# Autodesk Inventor assembly: A-02-0
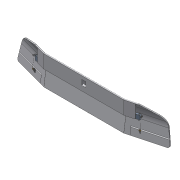
[picture p0: Inventor's stored thumbnail of the model, 180x180]
Saved by Autodesk Inventor 2019 (Build 230136000, 136)
## iProperties
Created: 2022-04-10
Part Number: A-02-0
Document SubType Name: Assembly
Designer: solyo
Mass: 70.6631 g
Surface Area: 2345.99 cm^2
Volume: 647.935 cm^3
Density: 0.109059 g/cm^3
Author: solyo
## Documents named in this file (11)
- D:\Modelling\RC\RC Trainer V1\ASSEMBLY\A-02-0-WING\A-02-0.iam
- D:\Modelling\RC\RC Trainer V1\Parts\PF-00-0-WING\PF-00-0-1.ipt
- D:\Modelling\RC\RC Trainer V1\Parts\C-03-0-SERVO_3G\C-03-0\CCW.ipt
- D:\Modelling\RC\RC Trainer V1\Parts\C-03-0-SERVO_3G\C-03-0\CW.ipt
- D:\Modelling\RC\RC Trainer V1\Parts\PP-00-0-CONTROL_HORN\PP-00-0-0.ipt
- D:\Modelling\RC\RC Trainer V1\PARTS\PM-00-0-PUSHROD\PM-00-0-0\AILERON.ipt
- D:\Modelling\RC\RC Trainer V1\Parts\C-04-0-SERVO_LINKAGE_STOPPER\C-04-0.ipt
- D:\Modelling\RC\RC Trainer V1\Parts\C-03-0-SERVO_3G\C-03-0.ipt
- D:\Modelling\RC\RC Trainer V1\PARTS\PM-00-0-PUSHROD\PM-00-0-0.ipt
- D:\Modelling\RC\RC Trainer V1\PARTS\PW-02-0-PIN\PW-02-0-0\GUARD.ipt
- D:\Modelling\RC\RC Trainer V1\PARTS\PW-02-0-PIN\PW-02-0-0.ipt
## Components (10 placed, 7 different names)
1. PF-00-0-1:1 — Mate:13, Mate:14
2. CCW:1 — Insert:4
3. CW:2
4. PP-00-0-0:1
5. PP-00-0-0:2
6. AILERON:1
7. C-04-0:1 — Mate:11
8. C-04-0:2
9. AILERON:2 — Insert:4, Mate:11
10. GUARD:1 — Mate:12, Mate:13, Mate:14
## Relationships (20: Mate 14, Insert 4, Flush 2)
- [Mate]: PF-00-0-1:1 ↔ CCW:1
- [Mate]: PF-00-0-1:1 ↔ CW:2
- [Mate]: PF-00-0-1:1 ↔ PP-00-0-0:1
- [Mate]: PF-00-0-1:1 ↔ PP-00-0-0:1
- [Mate]: PF-00-0-1:1 ↔ PP-00-0-0:2
- [Mate]: PF-00-0-1:1 ↔ PP-00-0-0:2
- [Mate]: CW:2 ↔ AILERON:1
- [Flush]: PF-00-0-1:1 ↔ CCW:1
- [Mate]: PF-00-0-1:1 ↔ CCW:1
- [Flush]: PF-00-0-1:1 ↔ CW:2
- [Mate]: PF-00-0-1:1 ↔ CW:2
- [Insert]: PP-00-0-0:2 ↔ C-04-0:1
- [Insert] (1 mm): CW:2 ↔ AILERON:1
- [Insert]: PP-00-0-0:1 ↔ C-04-0:2
- [Mate]: AILERON:1 ↔ C-04-0:2
- Insert:4 (1 mm): CCW:1 ↔ AILERON:2
- Mate:11: C-04-0:1 ↔ AILERON:2
- Mate:12: GUARD:1
- Mate:13: PF-00-0-1:1 ↔ GUARD:1
- Mate:14 (-2.5 mm): PF-00-0-1:1 ↔ GUARD:1
## Named parameters: d55_d6 = 0 mm, d58_d9 = 0 mm, d60_d11 = 0 mm, d61_d12 = 0 mm, d63_d14 = 0 mm, d67_d18 = 0 mm
